# Autodesk Inventor assembly: PeristalticPump
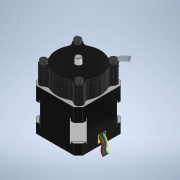
[picture p0: Inventor's stored thumbnail of the model, 180x180]
Saved by Autodesk Inventor 2020.2 (Build 242310000, 310)
## iProperties
Created: 2020-09-02
Part Number: PeristalticPump
Document SubType Name: Assembly
Designer: JK
Author: JK
## Documents named in this file (8)
- C:\Users\JK\Documents\Inventor\PeristalticPump\PeristalticPump.iam
- C:\Users\JK\Documents\Inventor\PeristalticPump\MOTOR.ipt
- C:\Users\JK\Documents\Inventor\PeristalticPump\Case.ipt
- C:\Users\JK\Documents\Inventor\PeristalticPump\M5DIN125Washer.ipt
- C:\Users\JK\Documents\Inventor\PeristalticPump\LidAssembly.iam
- C:\Users\JK\Documents\Inventor\PeristalticPump\ImpellerAssembly.iam
- C:\Users\JK\Documents\Inventor\PeristalticPump\Hose.ipt
- C:\Users\JK\Documents\Inventor\PeristalticPump\Casewithmount.ipt
## Components (7 placed, 7 different names)
1. MOTOR:1 — Mate:3, Mate:12, Mate:14, Mate:15, Angle:1, Mate:18, Angle:2
2. Case:1 — Mate:3, Mate:14, Mate:16, Mate:17
3. M5DIN125Washer:1 — Mate:12
4. LidAssembly:1 [sub-assembly] — Angle:1
5. ImpellerAssembly:1 [sub-assembly] — Mate:15
6. Hose:1 — Mate:16
7. Casewithmount:1 — Mate:17, Mate:18, Angle:2
## Relationships (14: Mate 12, Angle 2)
- [Mate]: MOTOR:1 ↔ ImpellerAssembly:1
- Mate:3: MOTOR:1 ↔ Case:1
- [Mate]: MOTOR:1 ↔ LidAssembly:1
- [Mate]: Case:1 ↔ LidAssembly:1
- [Mate]: Case:1 ↔ LidAssembly:1
- Mate:12: MOTOR:1 ↔ M5DIN125Washer:1
- [Mate]: M5DIN125Washer:1 ↔ ImpellerAssembly:1
- Mate:14: MOTOR:1 ↔ Case:1
- Mate:15 (5 mm): MOTOR:1 ↔ ImpellerAssembly:1
- Mate:16: Case:1 ↔ Hose:1
- Angle:1 (0 deg): MOTOR:1 ↔ LidAssembly:1
- Mate:17: Case:1 ↔ Casewithmount:1
- Mate:18: MOTOR:1 ↔ Casewithmount:1
- Angle:2 (0 deg): MOTOR:1 ↔ Casewithmount:1
